# Autodesk Inventor assembly: Wheel
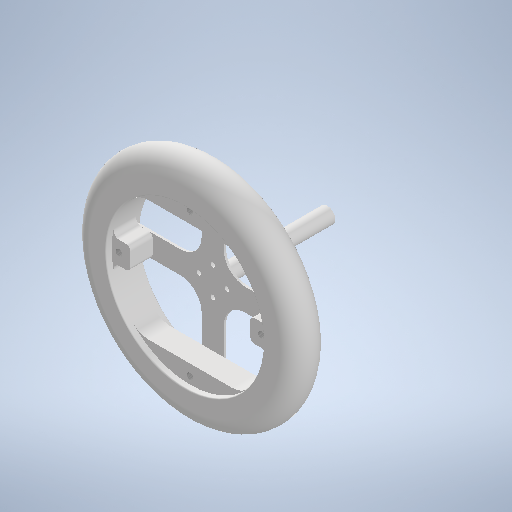
[picture p0: Inventor's stored thumbnail of the model, 512x512]
Saved by Autodesk Inventor 2025 (Build 290162000, 162)
## iProperties
Created: 2025-01-08
Part Number: Wheel
Document SubType Name: Assembly
Designer: 5014070
Author: 5014070
## Documents named in this file (5)
- C:\Users\5014070\Documents\GitHub\Mechanical\SeattleSolarCar2024-2025\Steering Wheel\Wheel.iam
- C:\Users\5014070\Documents\GitHub\Mechanical\SeattleSolarCar2024-2025\Steering Wheel\steering sheet.ipt
- C:\Users\5014070\Documents\GitHub\Mechanical\SeattleSolarCar2024-2025\Steering Wheel\steering wheel.ipt
- C:\Users\5014070\Documents\GitHub\Mechanical\SeattleSolarCar2024-2025\Steering Wheel\flange.ipt
- C:\Users\5014070\Documents\GitHub\Mechanical\SeattleSolarCar2024-2025\Steering Wheel\rod attachment(wheelside).ipt
## Components (4 placed, 4 different names)
1. steering sheet:1 — Mate:1, Mate:2, Mate:3, Mate:4, Mate:5, Mate:6, Mate:7
2. steering wheel:1 — Mate:1, Mate:2, Mate:3
3. flange:1 — Mate:4, Mate:5, Mate:6, Cylindrical:1
4. rod attachment(wheelside):1 — Mate:7, Cylindrical:1
## Relationships (8: Mate 7, CylindricalJoint 1)
- Mate:1: steering sheet:1 ↔ steering wheel:1
- Mate:2: steering sheet:1 ↔ steering wheel:1
- Mate:3: steering sheet:1 ↔ steering wheel:1
- Mate:4: steering sheet:1 ↔ flange:1
- Mate:5: steering sheet:1 ↔ flange:1
- Mate:6: steering sheet:1 ↔ flange:1
- Mate:7: steering sheet:1 ↔ rod attachment(wheelside):1
- Cylindrical:1: flange:1 ↔ rod attachment(wheelside):1
